# Autodesk Inventor assembly: inner
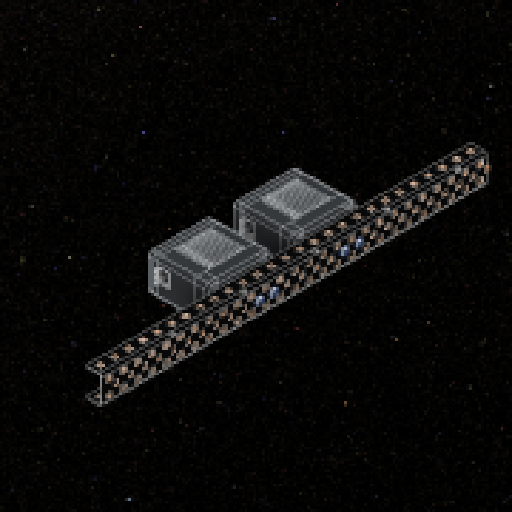
[picture p0: Inventor's stored thumbnail of the model, 512x512]
Saved by Autodesk Inventor 2024 (Build 280153000, 153)
## iProperties
Created: 2024-02-24
Part Number: inner
Document SubType Name: Assembly
Designer: Averey Ku
Author: Averey Ku
## Documents named in this file (4)
- D:\vex_robotics\hardware\cad\lil_zoom\chassis\drivebay\inner.iam
- D:\vex_robotics\hardware\cad\VEX-CAD-Inventor-1.41\Structure\C Channel\Aluminum 1x2x1\Alu C 1x2x1x27.ipt
- D:\vex_robotics\hardware\cad\VEX-CAD-Inventor-1.41\Electronics\Motors with Screws\SteelM-StarS.iam
- D:\vex_robotics\hardware\cad\VEX-CAD-Inventor-1.41\Electronics\Motors with Screws.iam
## Components (3 placed, 2 different names)
1. Alu C 1x2x1x27:1 — Insert:1, Mate:1, Insert:2, Mate:2
2. SteelM-StarS:1 [sub-assembly] — Insert:1, Mate:1
3. SteelM-StarS:2 [sub-assembly] — Insert:2, Mate:2
## Relationships (4: Insert 2, Mate 2)
- Insert:1: Alu C 1x2x1x27:1 ↔ SteelM-StarS:1
- Mate:1: Alu C 1x2x1x27:1 ↔ SteelM-StarS:1
- Insert:2: Alu C 1x2x1x27:1 ↔ SteelM-StarS:2
- Mate:2: Alu C 1x2x1x27:1 ↔ SteelM-StarS:2
